# Autodesk Inventor assembly: Double Acting Piston
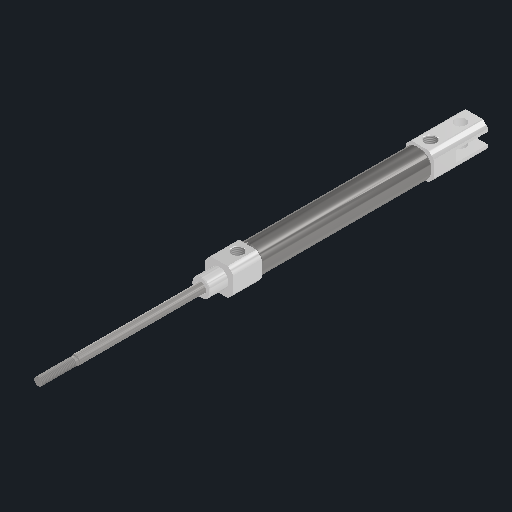
[picture p0: Inventor's stored thumbnail of the model, 512x512]
Saved by Autodesk Inventor 2023.4 (Build 274418000, 418)
## iProperties
Created: 2022-09-23
Part Number: Double Acting Piston
Document SubType Name: Assembly
Designer: maxxw
Mass: 9.29214 g
Surface Area: 91.0706 cm^2
Volume: 9.29214 cm^3
Author: maxxw
## Documents named in this file (3)
- C:\Users\Meer\OneDrive\Documents\GitHub\2024-599Z\Cad\Library\VEX-CAD-Inventor-1.4.0\Motion\Pneumatics\Double Acting Piston.iam
- C:\Users\Meer\OneDrive\Documents\GitHub\2024-599Z\Cad\Library\VEX-CAD-Inventor-1.4.0\Motion\Pneumatics\Reference Parts\Pistons\Double Acting Piston Body.ipt
- C:\Users\Meer\OneDrive\Documents\GitHub\2024-599Z\Cad\Library\VEX-CAD-Inventor-1.4.0\Motion\Pneumatics\Reference Parts\Pistons\Double Acting Piston Rod.ipt
## Components (2 placed, 2 different names)
1. Double Acting Piston Body:1 — Mate:1, Mate:2
2. Double Acting Piston Rod:1 — Mate:1, Mate:2
## Relationships (2: Mate 2)
- Mate:1: Double Acting Piston Body:1 ↔ Double Acting Piston Rod:1
- Mate:2: Double Acting Piston Body:1 ↔ Double Acting Piston Rod:1
